# Autodesk Inventor assembly: actuatorassembly
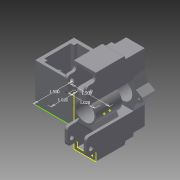
[picture p0: Inventor's stored thumbnail of the model, 180x180]
Saved by Autodesk Inventor 2013 SP2 (Build 170200200, 200)
## iProperties
Created: 2016-02-12
Part Number: actuatorassembly
Document SubType Name: Assembly
Designer: 2016ahoganso
Author: 2016ahoganso
## Documents named in this file (3)
- \\198.38.27.7\Senior\2016ahoganso\Robotics\actuatorassembly.iam
- \\198.38.27.7\Senior\2016ahoganso\Robotics\freeholder.ipt
- \\198.38.27.7\Senior\2016ahoganso\Robotics\actuatorholder.ipt
## Components (2 placed, 2 different names)
1. freeholder:1 — Mate:3, Flush:1
2. actuatorholder:1 — Mate:2, Mate:3, Flush:1
## Relationships (3: Mate 2, Flush 1)
- Mate:2: actuatorholder:1
- Mate:3: freeholder:1 ↔ actuatorholder:1
- Flush:1: freeholder:1 ↔ actuatorholder:1
